# Autodesk Inventor assembly: hopper final 1
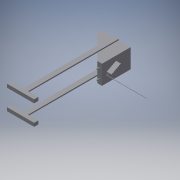
[picture p0: Inventor's stored thumbnail of the model, 180x180]
Saved by Autodesk Inventor 2019 (Build 230136000, 136)
## iProperties
Created: 2020-02-13
Part Number: hopper final 1
Document SubType Name: Assembly
Designer: ASUS
Author: ASUS
## Documents named in this file (4)
- F:\General\subsystem 1\hopper final 1.iam
- F:\General\subsystem 1\hopper 2.ipt
- F:\General\subsystem 1\Part2.ipt
- F:\General\subsystem 1\hopper stand.ipt
## Components (5 placed, 3 different names)
1. hopper 2:1 — Rigid:1, Rigid:2, Rigid:4
2. hopper 2:2 — Rigid:1, Rigid:3
3. Part2:1 — Rigid:2
4. hopper stand:1 — Rigid:4
5. hopper stand:2 — Rigid:3
## Relationships (4: WeldJoint 4)
- Rigid:1 [WeldJoint]: hopper 2:1 ↔ hopper 2:2
- Rigid:2 [WeldJoint]: hopper 2:1 ↔ Part2:1
- Rigid:3 [WeldJoint]: hopper 2:2 ↔ hopper stand:2
- Rigid:4 [WeldJoint]: hopper 2:1 ↔ hopper stand:1
